# Autodesk Inventor assembly: jst-vh-2p
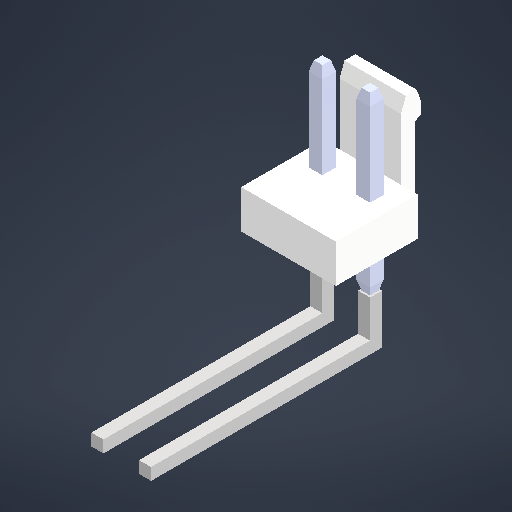
[picture p0: Inventor's stored thumbnail of the model, 512x512]
Saved by Autodesk Inventor 2025.2 (Build 292293000, 293)
## iProperties
Created: 2025-12-13
Part Number: jst-vh-2p
Document SubType Name: Assembly
Designer: sam
Author: sam
## iProperties of the stored document B2P-VH.iam
Created: 2023-12-10
Part Number: B2P-VH
Description: STEP AP214
Document SubType Name: Assembly
Designer: sam
Sending System: SolidWorks 2021
Preprocessor: SwSTEP 2.0
Title: B2P-VH.STEP
Revision Number: ANY
## iProperties of the stored document BxP-VH_2.ipt
Created: 2025-12-13
Part Number: BxP-VH_2
Material: Generic
Document SubType Name: Modeling
Designer: sam
Density: 1 g/cm^3
Appearance: Default
Author: sam
Revision Number: ANY
## iProperties of the stored document pin.ipt
Created: 2025-12-13
Part Number: pin
Material: Generic
Document SubType Name: Modeling
Designer: sam
Density: 1 g/cm^3
Appearance: Default
Author: sam
Revision Number: ANY
## Documents named in this file (7)
- G:\projects\primary\regulated-irrigation-system\model\asm\electronic-components\jst-vh-2p_short\jst-vh-2p_short-up.iam
- **G:\projects\primary\regulated-irrigation-system\model\asm\electronic-components\jst-vh-2p_short\jst-vh-2p_short-up.iam*LocalDocs*xAaaaqhaaAaaaaaaaAaaaa2kq5b*B2P-VH.iam
- G:\projects\primary\regulated-irrigation-system\model\asm\electronic-components\jst-vh-2p_short\jst-vh-2p_wire_short-up.ipt
- **G:\projects\primary\regulated-irrigation-system\model\asm\pcb\jst-vh-2p\jst-vh-2p.iam*LocalDocs*xAaaaqhaaAaaaaaaaAaaaa2kq5b*B2P-VH.iam
- **G:\projects\primary\regulated-irrigation-system\model\asm\pcb\jst-vh-2p\jst-vh-2p.iam*LocalDocs*xAaaaqfcaAaaaaaaaAaaaazwj0a*BxP-VH_2.ipt
- **G:\projects\primary\regulated-irrigation-system\model\asm\pcb\jst-vh-2p\jst-vh-2p.iam*LocalDocs*xAaaaqlcaAaaaaaaaAaaaqaiuDc*pin.ipt
- G:\docs\kicad-libraries\B2P-VH\B2P-VH.step
## Components (3 placed, 2 different names)
1. B2P-VH:1 [sub-assembly] — Mate:1, Mate:2, Flush:1, Flush:2, Flush:3, Flush:4
2. jst-vh-2p_wire_short-up:1 — Mate:1, Flush:2, Flush:3
3. jst-vh-2p_wire_short-up:2 — Mate:2, Flush:1, Flush:4
## Relationships (6: Flush 4, Mate 2)
- Mate:1: B2P-VH:1 ↔ jst-vh-2p_wire_short-up:1
- Mate:2: B2P-VH:1 ↔ jst-vh-2p_wire_short-up:2
- Flush:1 (0.07 mm): B2P-VH:1 ↔ jst-vh-2p_wire_short-up:2
- Flush:2 (0.07 mm): B2P-VH:1 ↔ jst-vh-2p_wire_short-up:1
- Flush:3 (0.07 mm): B2P-VH:1 ↔ jst-vh-2p_wire_short-up:1
- Flush:4 (0.07 mm): B2P-VH:1 ↔ jst-vh-2p_wire_short-up:2
